# Autodesk Inventor assembly: OmniBevelGear
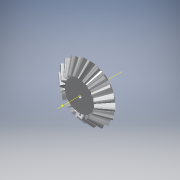
[picture p0: Inventor's stored thumbnail of the model, 180x180]
Saved by Autodesk Inventor 2016 (Build 200138000, 138)
## iProperties
Created: 2017-02-08
Part Number: OmniBevelGear
Document SubType Name: Assembly
Designer: Evan Phil George
Author: Evan Phil George
## Documents named in this file (2)
- C:\Users\Evan Phil George\Desktop\Ball Balancing Robot\TestBenchInventor\Transmission\OmniBevelGear.iam
- C:\Users\Evan Phil George\Desktop\Ball Balancing Robot\TestBenchInventor\Transmission\OmniBevelGear\Design Accelerator\Bevel Gears1.iam
## Components (1 placed, 1 different names)
1. Bevel Gears:1 [sub-assembly] — Mate:1, Mate:2
## Relationships (2: Mate 2)
- Mate:1: Bevel Gears:1
- Mate:2: Bevel Gears:1
